# Autodesk Inventor assembly: Loop Assembly
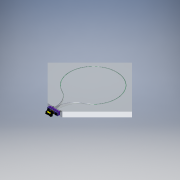
[picture p0: Inventor's stored thumbnail of the model, 180x180]
Saved by Autodesk Inventor 2016 (Build 200138000, 138)
## iProperties
Created: 2015-08-17
Part Number: Loop Assembly
Document SubType Name: Assembly
Designer: Cosmic
Author: Cosmic
## Documents named in this file (6)
- C:\Users\Jonathan\Documents\Projects\loop\scintillatorPanel\loopPanel.iam
- C:\Users\Jonathan\Documents\Projects\loop\scintillatorPanel\loopPanel.ipt
- C:\Users\Jonathan\Documents\Projects\loop\scintillatorPanel\fiberLoop.ipt
- C:\Users\Jonathan\Documents\Projects\loop\scintillatorPanel\dependency\mppcSensorInterface\cad\mppcSensor.iam
- C:\Users\Jonathan\Documents\Projects\loop\scintillatorPanel\hardware\4-40x0.5in.ipt
- C:\Users\Jonathan\Documents\Projects\loop\scintillatorPanel\Scintillator.xlsx
## Components (5 placed, 4 different names)
1. loopPanel:1 — Mate:1, Mate:2, Tangent:1, Mate:3, Mate:4, Mate:5, Mate:6, Angle:2
2. fiberLoop:1 — Mate:1, Mate:2, Tangent:1
3. mppcSensor:1 [sub-assembly] — Mate:3, Mate:4, Mate:5, Mate:7, Angle:1, Mate:8, Mate:9
4. 4-40x0.5in:1 — Mate:8, Mate:9, Angle:2
5. 4-40x0.5in:2 — Mate:6, Mate:7, Angle:1
## Relationships (12: Mate 9, Angle 2, Tangent 1)
- Mate:1: loopPanel:1 ↔ fiberLoop:1
- Mate:2: loopPanel:1 ↔ fiberLoop:1
- Tangent:1: loopPanel:1 ↔ fiberLoop:1
- Mate:3: loopPanel:1 ↔ mppcSensor:1
- Mate:4: loopPanel:1 ↔ mppcSensor:1
- Mate:5: loopPanel:1 ↔ mppcSensor:1
- Mate:6: loopPanel:1 ↔ 4-40x0.5in:2
- Mate:7: mppcSensor:1 ↔ 4-40x0.5in:2
- Angle:1 (0 deg): mppcSensor:1 ↔ 4-40x0.5in:2
- Mate:8: mppcSensor:1 ↔ 4-40x0.5in:1
- Mate:9: mppcSensor:1 ↔ 4-40x0.5in:1
- Angle:2 (0 deg): loopPanel:1 ↔ 4-40x0.5in:1
## Named parameters: OpticalFiberClearence = 0.15 mm, MPPCClearence = 0.075 mm, FiberSensorClerence = 0.5 mm, OpticalFiberDiameter = 1 mm, ScintillatorThickness = 12.7 mm, SmallTrackDiameter = 175 mm, LargeTrackRatio = 3, ScintillatorEdgeClearence = 3 mm, ScintillatorWidth = 146.05 mm, ScintillatorHeight = 146.05 mm, ShallowTrackDepth = 1.2 mm, MPPCSensorClearence = 1.45 mm, MPPCSensorOffsett = 2.105 mm, MPPCWidth = 5.9 mm, MPPCHeight = 6.55 mm, FiberEdgeOffsett = 5 mm, MPPCDepth = 1 mm, LongFiberAngle = 30 deg, ShortFiberAngle = 78 deg, LoopLargeTrackRatio = 1.25, LoopSmallTrackDiameter = 90 mm, MountingScrewDepth = 4 mm, MountingScrewOffsett = 9 mm, LoopLength = 140 mm, CornerCut = 25.4 mm, FiberSensorClerance = 0.5 mm, DeepTrackDepth = 6.95 mm, OpticalFiberClearance = 0.1 mm, ScintillatorEdgeClearance = 3 mm
